# Autodesk Inventor assembly: Nema17MetGearbox
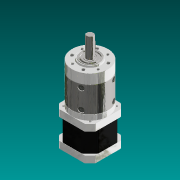
[picture p0: Inventor's stored thumbnail of the model, 180x180]
Saved by Autodesk Inventor 2020.2 (Build 242310000, 310)
## iProperties
Created: 2020-05-14
Part Number: Nema17MetGearbox
Document SubType Name: Assembly
Designer: Svend
Author: Svend
## Documents named in this file (3)
- C:\Users\Svend\OneDrive\Documents\GitHub\BeerMinder\3D-model\Nema17MetGearbox.iam
- C:\Users\Svend\OneDrive\Documents\GitHub\BeerMinder\3D-model\stepper motors\42BYG Stepper Motor.ipt
- C:\Users\Svend\OneDrive\Documents\GitHub\BeerMinder\3D-model\gearbox\gearbox.iam
## Components (2 placed, 2 different names)
1. 42BYG Stepper Motor:1 — Mate:1, Mate:2
2. gearbox:1 [sub-assembly] — Mate:1, Mate:2
## Relationships (2: Mate 2)
- Mate:1: 42BYG Stepper Motor:1 ↔ gearbox:1
- Mate:2: 42BYG Stepper Motor:1 ↔ gearbox:1
